# Autodesk Inventor assembly: COTS_WCP-0879_InlineClampingBearingBlock
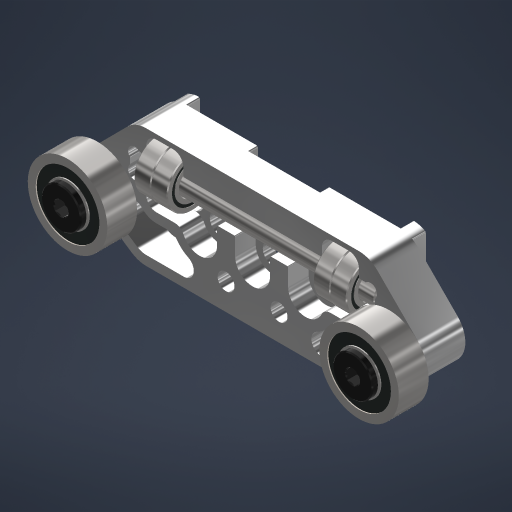
[picture p0: Inventor's stored thumbnail of the model, 512x512]
Saved by Autodesk Inventor 2024.3 (Build 283343000, 343)
## iProperties
Created: 2025-07-14
Part Number: COTS_WCP-0879_InlineClampingBearingBlock
Document SubType Name: Assembly
Designer: Kenji
Author: Kenji
## Documents named in this file (6)
- C:\Users\Kenji\Documents\GitHub\1622-2025-Reefscape-Offseason\COTS Library\Motion\Bearings\COTS_WCP-0879_InlineClampingBearingBlock.iam
- C:\Users\Kenji\Documents\GitHub\1622-2025-Reefscape-Offseason\COTS Library\Motion\Bearings\WCP-0897 (3)\WCP-0897 (3)\WCP-0212_0_250_radial_bearing.ipt
- C:\Users\Kenji\Documents\GitHub\1622-2025-Reefscape-Offseason\COTS Library\Motion\Bearings\WCP-0897 (3)\WCP-0897 (3)\WCP-0473 Rev1.ipt
- C:\Users\Kenji\Documents\GitHub\1622-2025-Reefscape-Offseason\COTS Library\Motion\Bearings\WCP-0897 (3)\WCP-0897 (3)\WCP-0498 Rev1.ipt
- C:\Users\Kenji\Documents\GitHub\1622-2025-Reefscape-Offseason\COTS Library\Motion\Bearings\WCP-0897 (3)\WCP-0897 (3)\WCP-0897-001 Rev1.ipt
- C:\Users\Kenji\Documents\GitHub\1622-2025-Reefscape-Offseason\COTS Library\Motion\Bearings\WCP-0897 (3)\WCP-0897 (3)\WCP-0897-002 Rev1.ipt
## Components (10 placed, 5 different names)
1. WCP-0212_0_250_radial_bearing:1 — Mate:11, Mate:12, Mate:13
2. WCP-0473 Rev1:1 — Mate:10, Mate:11, Mate:13
3. WCP-0498 Rev1:1 — Mate:2, Mate:3, Mate:18
4. WCP-0897-001 Rev1:1 — Tangent:1, Tangent:2, Mate:1, Mate:3, Mate:7, Mate:10, Mate:12, Mate:14, Mate:17
5. WCP-0897-002 Rev1:1 — Tangent:1, Tangent:2, Mate:1, Mate:2, Mate:4, Mate:5, Mate:6
6. WCP-0498 Rev1:2 — Mate:5, Mate:7, Mate:8
7. WCP-0498 Rev1:3 — Mate:4, Mate:18
8. WCP-0498 Rev1:4 — Mate:6, Mate:8
9. WCP-0473 Rev1:2 — Mate:14, Mate:15, Mate:16
10. WCP-0212_0_250_radial_bearing:2 — Mate:15, Mate:16, Mate:17
## Relationships (19: Mate 17, Tangent 2)
- Tangent:1: WCP-0897-001 Rev1:1 ↔ WCP-0897-002 Rev1:1
- Tangent:2: WCP-0897-001 Rev1:1 ↔ WCP-0897-002 Rev1:1
- Mate:1: WCP-0897-001 Rev1:1 ↔ WCP-0897-002 Rev1:1
- Mate:2: WCP-0498 Rev1:1 ↔ WCP-0897-002 Rev1:1
- Mate:3: WCP-0498 Rev1:1 ↔ WCP-0897-001 Rev1:1
- Mate:4: WCP-0897-002 Rev1:1 ↔ WCP-0498 Rev1:3
- Mate:5: WCP-0897-002 Rev1:1 ↔ WCP-0498 Rev1:2
- Mate:6: WCP-0897-002 Rev1:1 ↔ WCP-0498 Rev1:4
- Mate:7: WCP-0897-001 Rev1:1 ↔ WCP-0498 Rev1:2
- Mate:8: WCP-0498 Rev1:2 ↔ WCP-0498 Rev1:4
- Mate:10: WCP-0473 Rev1:1 ↔ WCP-0897-001 Rev1:1
- Mate:11: WCP-0212_0_250_radial_bearing:1 ↔ WCP-0473 Rev1:1
- Mate:12: WCP-0212_0_250_radial_bearing:1 ↔ WCP-0897-001 Rev1:1
- Mate:13: WCP-0212_0_250_radial_bearing:1 ↔ WCP-0473 Rev1:1
- Mate:14: WCP-0897-001 Rev1:1 ↔ WCP-0473 Rev1:2
- Mate:15: WCP-0473 Rev1:2 ↔ WCP-0212_0_250_radial_bearing:2
- Mate:16: WCP-0473 Rev1:2 ↔ WCP-0212_0_250_radial_bearing:2
- Mate:17: WCP-0897-001 Rev1:1 ↔ WCP-0212_0_250_radial_bearing:2
- Mate:18: WCP-0498 Rev1:1 ↔ WCP-0498 Rev1:3
